# Autodesk Inventor assembly: BallOnBeamDc
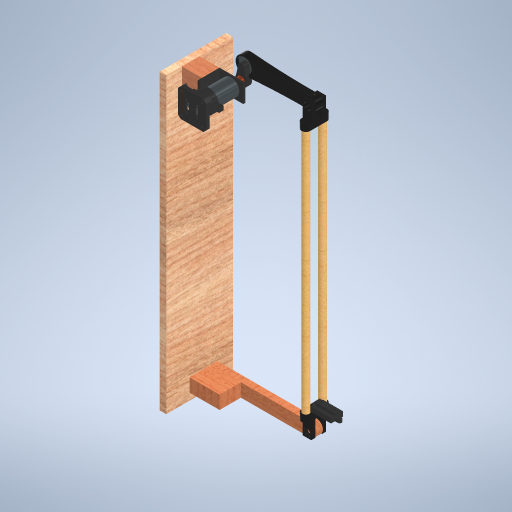
[picture p0: Inventor's stored thumbnail of the model, 512x512]
Saved by Autodesk Inventor 2023 (Build 270158000, 158)
## iProperties
Created: 2024-02-23
Part Number: BallOnBeamDc
Document SubType Name: Assembly
Designer: phili
Author: phili
## Documents named in this file (17)
- C:\Users\phili\FAUbox\Philipp\Bauprojekte\Ball_On_Beam\CAD\BallOnBeamDc.iam
- C:\Users\phili\FAUbox\Philipp\Bauprojekte\Ball_On_Beam\CAD\Bauteile\Grundfläche.ipt
- C:\Users\phili\FAUbox\Philipp\Bauprojekte\Ball_On_Beam\CAD\Bauteile\MotorBlock.ipt
- C:\Users\phili\FAUbox\Philipp\Bauprojekte\Ball_On_Beam\CAD\Bauteile\MotorHalterNeu.ipt
- C:\Users\phili\FAUbox\Philipp\Bauprojekte\Ball_On_Beam\CAD\Bauteile\DcMotor.ipt
- C:\Users\phili\FAUbox\Philipp\Bauprojekte\Ball_On_Beam\CAD\Bauteile\MotorAdapter.ipt
- C:\Users\phili\FAUbox\Philipp\Bauprojekte\Ball_On_Beam\CAD\Bauteile\MotorAnkerNeu.ipt
- C:\Users\phili\FAUbox\Philipp\Bauprojekte\Ball_On_Beam\CAD\Bauteile\Kugellager.ipt
- C:\Users\phili\FAUbox\Philipp\Bauprojekte\Ball_On_Beam\CAD\Bauteile\Hebel.ipt
- C:\Users\phili\FAUbox\Philipp\Bauprojekte\Ball_On_Beam\CAD\Bauteile\ObenMotor.ipt
- C:\Users\phili\FAUbox\Philipp\Bauprojekte\Ball_On_Beam\CAD\Bauteile\Stab.ipt
- C:\Users\phili\FAUbox\Philipp\Bauprojekte\Ball_On_Beam\CAD\Bauteile\HolzHalter.ipt
- C:\Users\phili\FAUbox\Philipp\Bauprojekte\Ball_On_Beam\CAD\Bauteile\HolzHalterNeu.ipt
- C:\Users\phili\FAUbox\Philipp\Bauprojekte\Ball_On_Beam\CAD\Bauteile\EncoderHalter.ipt
- C:\Users\phili\FAUbox\Philipp\Bauprojekte\Ball_On_Beam\CAD\Bauteile\SensorHalterSchale.ipt
- C:\Users\phili\FAUbox\Philipp\Bauprojekte\Ball_On_Beam\CAD\Bauteile\klemme.ipt
- C:\Users\phili\FAUbox\Philipp\Bauprojekte\Ball_On_Beam\CAD\Bauteile\InfraSensor.ipt
## Components (18 placed, 16 different names)
1. Grundfläche:1 — Fluchtend:1, Passend:1, Fluchtend:2, Passend:19, Fluchtend:6, Passend:27, Winkel:8, Winkel:9
2. MotorBlock:1 — Fluchtend:1, Passend:1, Fluchtend:2, Passend:2, Fluchtend:3, Fluchtend:4, Winkel:3
3. MotorHalterNeu:1 — Passend:2, Fluchtend:3, Fluchtend:4, Passend:3, Passend:4, Winkel:1, Passend:6, Winkel:2
4. DcMotor:1 — Passend:3, Passend:4, Winkel:1, Passend:5, Passend:29, Passend:30, Passend:31, Passend:34
5. MotorAdapter:1 — Passend:5, Passend:6, Winkel:2, Passend:7, Passend:8, Passend:9
6. MotorAnkerNeu:1 — Passend:7, Passend:8, Passend:9, Passend:10, Passend:11
7. Kugellager:1 — Passend:10, Passend:11, Passend:12, Fluchtend:5, Winkel:7
8. Hebel:1 — Passend:12, Fluchtend:5, Winkel:3, Passend:13, Passend:14, Winkel:4, Winkel:7
9. ObenMotor:1 — Passend:13, Passend:14, Winkel:4, Passend:23, Passend:24, Passend:25
10. HolzHalter:1 — Passend:19, Fluchtend:6, Passend:21, Passend:22, Passend:28, Fluchtend:7, Winkel:10
11. ObenMotor:2 — Passend:21, Passend:22, Passend:26, Passend:36, Passend:37, Passend:38, Passend:39
12. Stab:1 — Passend:23, Passend:24, Passend:25, Passend:26
13. HolzHalterNeu:1 — Passend:27, Passend:28, Fluchtend:7
14. EncoderHalter:1 — Passend:29, Passend:30, Winkel:8, Passend:32, Passend:33
15. SensorHalterSchale:1 — Passend:31, Passend:32, Passend:33, Passend:35
16. klemme:1 — Passend:34, Passend:35
17. Stab:2 — Passend:36, Passend:37, Winkel:9
18. InfraSensor:1 — Passend:38, Passend:39, Winkel:10
## Relationships (49: Mate 34, Angle 8, Flush 7)
- Fluchtend:1 [Flush]: Grundfläche:1 ↔ MotorBlock:1
- Passend:1 [Mate]: Grundfläche:1 ↔ MotorBlock:1
- Fluchtend:2 [Flush] (-50 mm): Grundfläche:1 ↔ MotorBlock:1
- Passend:2 [Mate]: MotorBlock:1 ↔ MotorHalterNeu:1
- Fluchtend:3 [Flush]: MotorBlock:1 ↔ MotorHalterNeu:1
- Fluchtend:4 [Flush]: MotorBlock:1 ↔ MotorHalterNeu:1
- Passend:3 [Mate]: MotorHalterNeu:1 ↔ DcMotor:1
- Passend:4 [Mate]: MotorHalterNeu:1 ↔ DcMotor:1
- Winkel:1 [Angle] (0 deg): MotorHalterNeu:1 ↔ DcMotor:1
- Passend:5 [Mate]: DcMotor:1 ↔ MotorAdapter:1
- Passend:6 [Mate]: MotorHalterNeu:1 ↔ MotorAdapter:1
- Winkel:2 [Angle] (90 deg): MotorHalterNeu:1 ↔ MotorAdapter:1
- Passend:7 [Mate]: MotorAdapter:1 ↔ MotorAnkerNeu:1
- Passend:8 [Mate]: MotorAdapter:1 ↔ MotorAnkerNeu:1
- Passend:9 [Mate]: MotorAdapter:1 ↔ MotorAnkerNeu:1
- Passend:10 [Mate]: MotorAnkerNeu:1 ↔ Kugellager:1
- Passend:11 [Mate]: MotorAnkerNeu:1 ↔ Kugellager:1
- Passend:12 [Mate]: Kugellager:1 ↔ Hebel:1
- Fluchtend:5 [Flush]: Kugellager:1 ↔ Hebel:1
- Winkel:3 [Angle] (180 deg): MotorBlock:1 ↔ Hebel:1
- Passend:13 [Mate]: Hebel:1 ↔ ObenMotor:1
- Passend:14 [Mate]: Hebel:1 ↔ ObenMotor:1
- Winkel:4 [Angle] (-90 deg): Hebel:1 ↔ ObenMotor:1
- Passend:19 [Mate]: Grundfläche:1 ↔ HolzHalter:1
- Fluchtend:6 [Flush] (23 mm): Grundfläche:1 ↔ HolzHalter:1
- Winkel:7 [Angle] (0 deg): Kugellager:1 ↔ Hebel:1
- Passend:21 [Mate]: HolzHalter:1 ↔ ObenMotor:2
- Passend:22 [Mate]: HolzHalter:1 ↔ ObenMotor:2
- Passend:23 [Mate]: ObenMotor:1 ↔ Stab:1
- Passend:24 [Mate]: ObenMotor:1 ↔ Stab:1
- Passend:25 [Mate]: ObenMotor:1 ↔ Stab:1
- Passend:26 [Mate]: ObenMotor:2 ↔ Stab:1
- Passend:27 [Mate]: Grundfläche:1 ↔ HolzHalterNeu:1
- Passend:28 [Mate]: HolzHalter:1 ↔ HolzHalterNeu:1
- Fluchtend:7 [Flush]: HolzHalter:1 ↔ HolzHalterNeu:1
- Passend:29 [Mate]: DcMotor:1 ↔ EncoderHalter:1
- Passend:30 [Mate]: DcMotor:1 ↔ EncoderHalter:1
- Winkel:8 [Angle] (0 deg): Grundfläche:1 ↔ EncoderHalter:1
- Passend:31 [Mate]: DcMotor:1 ↔ SensorHalterSchale:1
- Passend:32 [Mate]: EncoderHalter:1 ↔ SensorHalterSchale:1
- Passend:33 [Mate]: EncoderHalter:1 ↔ SensorHalterSchale:1
- Passend:34 [Mate]: DcMotor:1 ↔ klemme:1
- Passend:35 [Mate]: SensorHalterSchale:1 ↔ klemme:1
- Passend:36 [Mate]: ObenMotor:2 ↔ Stab:2
- Passend:37 [Mate]: ObenMotor:2 ↔ Stab:2
- Winkel:9 [Angle] (0 deg): Grundfläche:1 ↔ Stab:2
- Passend:38 [Mate]: ObenMotor:2 ↔ InfraSensor:1
- Passend:39 [Mate]: ObenMotor:2 ↔ InfraSensor:1
- Winkel:10 [Angle] (0 deg): HolzHalter:1 ↔ InfraSensor:1
